# Autodesk Inventor assembly: Box
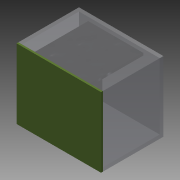
[picture p0: Inventor's stored thumbnail of the model, 180x180]
Saved by Autodesk Inventor 2013 (Build 170138000, 138)
## iProperties
Created: 2013-06-27
Part Number: Box
Document SubType Name: Assembly
Designer: Kyle
Author: Kyle
## Documents named in this file (4)
- C:\Users\Kyle\Documents\Autodesk\Inventor\Projects\ROV\Box\Box.iam
- C:\Users\Kyle\Documents\Autodesk\Inventor\Projects\ROV\Box\Box Bottom.ipt
- C:\Users\Kyle\Documents\Autodesk\Inventor\Projects\ROV\Box\Box Cover.ipt
- C:\Users\Kyle\Documents\Autodesk\Inventor\Projects\ROV\Box\Camera.ipt
## Components (3 placed, 3 different names)
1. Box Bottom:1 — Mate:1, Flush:1, Mate:2, Flush:2, Mate:3, Flush:3
2. Box Cover:1 — Mate:1, Flush:1, Flush:3
3. Camera:1 — Mate:2, Flush:2, Mate:3
## Relationships (6: Mate 3, Flush 3)
- Mate:1: Box Bottom:1 ↔ Box Cover:1
- Flush:1: Box Bottom:1 ↔ Box Cover:1
- Mate:2: Box Bottom:1 ↔ Camera:1
- Flush:2: Box Bottom:1 ↔ Camera:1
- Mate:3 (8.89 mm): Box Bottom:1 ↔ Camera:1
- Flush:3: Box Bottom:1 ↔ Box Cover:1
